# Autodesk Inventor assembly: Robot
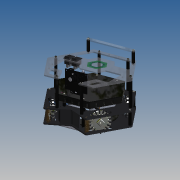
[picture p0: Inventor's stored thumbnail of the model, 180x180]
Saved by Autodesk Inventor 2017 (Build 210142000, 142)
## iProperties
Created: 2016-10-01
Part Number: Robot
Document SubType Name: Assembly
Designer: James Yelland
Author: James Yelland
## Documents named in this file (33)
- C:\Users\yella\git\LJ-STAND\Design\Models\Robot\Robot.iam
- C:\Users\yella\git\LJ-STAND\Design\Models\Robot\Bottom Plate.ipt
- C:\Users\yella\git\LJ-STAND\Design\Models\Robot\Motor Mount.ipt
- C:\Users\yella\git\LJ-STAND\Design\Models\Fasteners\Standoff 30 F-F.ipt
- C:\Users\yella\git\LJ-STAND\Design\Models\Fasteners\M3x10 Screw.ipt
- C:\Users\yella\git\LJ-STAND\Design\Models\Fasteners\M3 Hex Nut.ipt
- C:\Users\yella\git\LJ-STAND\Design\Models\Common\Imported Components\maxon_PN_0_1\maxon_PN_0_1.iam
- C:\Users\yella\git\LJ-STAND\Design\Models\Fasteners\M2x4 Screw.ipt
- C:\Users\yella\git\LJ-STAND\Design\Models\Robot\Light Sensor PCB.ipt
- C:\Users\yella\git\LJ-STAND\Design\Models\Common\Wheel.ipt
- C:\Users\yella\git\LJ-STAND\Design\Models\Robot\Middle Plate.ipt
- C:\Users\yella\git\LJ-STAND\Design\Models\Robot\TSOP Cover Ring.ipt
- C:\Users\yella\git\LJ-STAND\Design\Models\Robot\Main PCB.ipt
- C:\Users\yella\git\LJ-STAND\Design\Models\Fasteners\M3x20 Screw.ipt
- C:\Users\yella\git\LJ-STAND\Design\Models\Common\Pixy angle bracket.ipt
- C:\Users\yella\git\LJ-STAND\Design\Models\Pixy\pixy\Imported Components\Pixy(CMUcam5)\Pixy(CMUcam5).iam
- C:\Users\yella\git\LJ-STAND\Design\Models\Fasteners\Standoff 65 M-F.ipt
- C:\Users\yella\git\LJ-STAND\Design\Models\Robot\Top Plate.ipt
- C:\Users\yella\git\LJ-STAND\Design\Models\Robot\Handle.ipt
- C:\Users\yella\git\LJ-STAND\Design\Models\Common\Rocker switch.ipt
- C:\Users\yella\git\LJ-STAND\Design\Models\Fasteners\Standoff 25 F-F.ipt
- C:\Users\yella\git\LJ-STAND\Design\Models\Robot\Sonar Mount.ipt
- C:\Users\yella\git\LJ-STAND\Design\Models\Fasteners\M3x6 Screw.ipt
- C:\Users\yella\git\LJ-STAND\Design\Models\Common\Sonar.ipt
- C:\Users\yella\git\LJ-STAND\Design\Models\Robot\Light Sensor Cover.ipt
- C:\Users\yella\git\LJ-STAND\Design\Models\Robot\Motor sleeve.ipt
- C:\Users\yella\git\LJ-STAND\Design\Models\Robot\Laser Mount Plate.ipt
- C:\Users\yella\git\LJ-STAND\Design\Models\Robot\LDR Mount Plate.ipt
- C:\Users\yella\git\LJ-STAND\Design\Models\Robot\Light gate compression plate.ipt
- C:\Users\yella\git\LJ-STAND\Design\Models\Fasteners\Standoff 10 M-F.ipt
- C:\Users\yella\git\LJ-STAND\Design\Models\Common\XBee mount.ipt
- C:\Users\yella\git\LJ-STAND\Design\Models\Robot\Light sensor ball guard.ipt
- C:\Users\yella\git\LJ-STAND\Design\Models\Robot\Ball Capture Zone Cover.ipt
## Components (118 placed, 32 different names)
1. Bottom Plate:1 — Insert:1, Insert:2, Insert:3, Insert:4, Insert:5, Insert:6, Insert:7, Insert:8, Insert:35, Insert:36, Insert:37, Insert:38, Insert:39, Insert:40, Mate:27, Mate:28, Mate:29, Mate:30, Mate:31, Mate:32, Mate:33, Mate:34, Mate:35, Mate:36, Mate:37, Mate:38, Mate:40, Mate:41, Mate:42, Mate:43, Mate:44, Mate:45, Insert:197, Insert:198, Insert:199, Insert:206, Insert:207, Insert:208, Insert:209
2. Motor Mount:1 — Insert:15, Mate:13, Insert:25, Insert:26, Insert:27, Mate:33, Mate:34, Mate:35
3. Motor Mount:2 — Insert:16, Mate:14, Insert:22, Insert:23, Insert:24, Mate:27, Mate:28, Mate:29
4. Motor Mount:3 — Insert:18, Mate:15, Insert:19, Insert:20, Insert:21, Mate:36, Mate:37, Mate:38
5. Motor Mount:4 — Insert:17, Mate:16, Insert:28, Insert:29, Insert:30, Mate:30, Mate:31, Mate:32
6. Standoff 30 F-F:1 — Insert:3
7. Standoff 30 F-F:2 — Insert:4
8. Standoff 30 F-F:3 — Insert:2, Insert:50, Insert:127
9. Standoff 30 F-F:4 — Insert:1, Insert:49, Insert:126
10. M3x10 Screw:1 — Insert:5
11. M3x10 Screw:2 — Insert:7
12. M3x10 Screw:3 — Insert:6
13. M3x10 Screw:4 — Insert:8
14. maxon_PN_0_1:1 [sub-assembly] — Insert:16, Mate:14, Mate:18, Flush:2, Insert:184, Angle:3
15. maxon_PN_0_1:2 [sub-assembly] — Insert:17, Mate:16, Mate:20, Flush:4
16. maxon_PN_0_1:3 [sub-assembly] — Insert:15, Mate:13, Mate:19, Flush:3
17. maxon_PN_0_1:4 [sub-assembly] — Insert:18, Mate:15, Mate:17, Flush:1
18. M2x4 Screw:1 — Insert:25
19. M2x4 Screw:3 — Insert:19
20. M2x4 Screw:4 — Insert:28
21. M2x4 Screw:5 — Insert:27
22. M2x4 Screw:6 — Insert:26
23. M2x4 Screw:7 — Insert:24
24. M2x4 Screw:8 — Insert:21
25. M2x4 Screw:9 — Insert:20
26. M2x4 Screw:10 — Insert:29
27. M2x4 Screw:11 — Insert:23
28. M2x4 Screw:12 — Insert:22
29. M2x4 Screw:13 — Insert:30
30. Light Sensor PCB:1 — Insert:35, Insert:36, Insert:41, Insert:42, Insert:43, Insert:44
31. M3 Hex Nut:3 — Insert:41
32. M3x10 Screw:7 — Insert:37
33. M3 Hex Nut:4 — Insert:42, Insert:182
34. M3x10 Screw:8 — Insert:38
35. M3 Hex Nut:5 — Insert:43, Insert:183
36. M3x10 Screw:9 — Insert:39
37. M3 Hex Nut:6 — Insert:44
38. M3x10 Screw:10 — Insert:40
39. Wheel:1 — Mate:18, Flush:2
40. Wheel:2 — Mate:19, Flush:3
41. Wheel:3 — Mate:17, Flush:1
42. Wheel:4 — Mate:20, Flush:4
43. Middle Plate:1 — Insert:49, Insert:50, Insert:102, Insert:103, Insert:104, Insert:105, Insert:106, Insert:107, Insert:120, Insert:121, Insert:122, Insert:123, Insert:124, Insert:125, Insert:126, Insert:127, Insert:128, Insert:129, Insert:130, Insert:131, Insert:191, Insert:192, Insert:193, Insert:194
44. TSOP Cover Ring:1 — Insert:69, Insert:70, Angle:1, Angle:2, Insert:195, Insert:196
45. Main PCB:1 — Insert:69, Insert:70, Insert:71, Insert:72, Insert:73, Insert:74, Insert:94, Insert:95
46. M3x20 Screw:1 — Insert:74
47. M3x20 Screw:2 — Insert:73
48. M3x20 Screw:3 — Insert:72
49. M3x20 Screw:4 — Insert:71
50. Pixy angle bracket:1 — Insert:95, Angle:2, Insert:168
51. Pixy angle bracket:2 — Insert:94, Angle:1, Insert:169
52. Pixy(CMUcam5):1 [sub-assembly] — Insert:168, Insert:169
53. Standoff 65 M-F:3 — Insert:102
54. Standoff 65 M-F:4 — Insert:103, Insert:140
55. Standoff 65 M-F:5 — Insert:106
56. Standoff 65 M-F:6 — Insert:107
57. Standoff 65 M-F:7 — Insert:105, Insert:141
58. Standoff 65 M-F:8 — Insert:104
59. Handle:1 — Insert:136, Insert:137, Insert:138, Insert:139
60. M3x10 Screw:19 — Insert:120
61. M3x10 Screw:20 — Insert:122
62. M3 Hex Nut:17 — Insert:146
63. M3x10 Screw:21 — Insert:125
64. M3 Hex Nut:18 — Insert:144
65. M3x10 Screw:22 — Insert:124
66. M3 Hex Nut:19 — Insert:151
67. M3x10 Screw:23 — Insert:123
68. M3 Hex Nut:20 — Insert:150
69. M3x10 Screw:24 — Insert:121
70. Rocker switch:1 — Mate:21, Mate:22, Mate:23
71. Rocker switch:2 — Mate:24, Mate:25, Mate:26
72. M3x10 Screw:25 — Insert:131
73. M3x10 Screw:26 — Insert:130
74. M3x10 Screw:27 — Insert:129
75. M3x10 Screw:28 — Insert:128
76. Standoff 25 F-F:1 — Insert:137, Insert:143
77. Standoff 25 F-F:2 — Insert:136, Insert:142
78. M3x10 Screw:29 — Insert:149
79. M3x10 Screw:30 — Insert:145
80. M3x10 Screw:31 — Insert:139
81. M3x10 Screw:32 — Insert:138
82. M3 Hex Nut:21 — Insert:147
83. M3 Hex Nut:22 — Insert:148
84. Sonar Mount:1 — Insert:156, Insert:157, Insert:170, Insert:171
85. Sonar Mount:2 — Insert:158, Insert:159, Insert:172, Insert:173
86. Sonar Mount:3 — Insert:152, Insert:153, Insert:176, Insert:177
87. Sonar Mount:4 — Insert:154, Insert:155, Insert:174, Insert:175
88. Top Plate:1 — Insert:140, Insert:141, Insert:142, Insert:143, Insert:144, Insert:145, Insert:146, Insert:147, Insert:148, Insert:149, Insert:150, Insert:151, Insert:152, Insert:153, Insert:154, Insert:155, Mate:21, Mate:22, Mate:23, Mate:24, Mate:25, Mate:26, Insert:156, Insert:157, Insert:158, Insert:159, Insert:160, Insert:161, Insert:162, Insert:163, Insert:164, Insert:165, Insert:166, Insert:167
89. M3x6 Screw:1 — Insert:160
90. M3x6 Screw:2 — Insert:161
91. M3x6 Screw:3 — Insert:162
92. M3x6 Screw:4 — Insert:167
93. M3x6 Screw:5 — Insert:163
94. M3x6 Screw:6 — Insert:165
95. M3x6 Screw:7 — Insert:166
96. M3x6 Screw:8 — Insert:164
97. Sonar:1 — Insert:176, Insert:177
98. Sonar:2 — Insert:174, Insert:175
99. Sonar:3 — Insert:172, Insert:173
100. Sonar:4 — Insert:170, Insert:171
101. Light Sensor Cover:1 — Insert:182, Insert:183
102. Motor sleeve:1 — Insert:184, Angle:3
103. Laser Mount Plate:1 — Mate:40, Mate:41, Mate:42, Insert:185, Insert:186
104. LDR Mount Plate:1 — Mate:43, Mate:44, Mate:45, Insert:187, Insert:188
105. Light gate compression plate:1 — Insert:185, Insert:186
106. Light gate compression plate:2 — Insert:187, Insert:188
107. Standoff 10 M-F:1 — Insert:191, Insert:196
108. Standoff 10 M-F:2 — Insert:194
109. Standoff 10 M-F:3 — Insert:193
110. Standoff 10 M-F:4 — Insert:192, Insert:195
111. XBee mount:1 — Insert:200, Insert:201
112. Standoff 10 M-F:5 — Insert:197, Insert:201
113. Standoff 10 M-F:6 — Insert:199
114. Standoff 10 M-F:7 — Insert:198, Insert:200
115. Standoff 25 F-F:3
116. Standoff 25 F-F:4
117. Light sensor ball guard:1 — Insert:206, Insert:207
118. Ball Capture Zone Cover:1 — Insert:208, Insert:209
## Relationships (165: Insert 126, Mate 32, Flush 4, Angle 3)
- Insert:1: Bottom Plate:1 ↔ Standoff 30 F-F:4
- Insert:2: Bottom Plate:1 ↔ Standoff 30 F-F:3
- Insert:3: Bottom Plate:1 ↔ Standoff 30 F-F:1
- Insert:4: Bottom Plate:1 ↔ Standoff 30 F-F:2
- Insert:5: Bottom Plate:1 ↔ M3x10 Screw:1
- Insert:6: Bottom Plate:1 ↔ M3x10 Screw:3
- Insert:7: Bottom Plate:1 ↔ M3x10 Screw:2
- Insert:8: Bottom Plate:1 ↔ M3x10 Screw:4
- Insert:15: Motor Mount:1 ↔ maxon_PN_0_1:3
- Insert:16: Motor Mount:2 ↔ maxon_PN_0_1:1
- Insert:17: Motor Mount:4 ↔ maxon_PN_0_1:2
- Insert:18: Motor Mount:3 ↔ maxon_PN_0_1:4
- Mate:13: Motor Mount:1 ↔ maxon_PN_0_1:3
- Mate:14: Motor Mount:2 ↔ maxon_PN_0_1:1
- Mate:15: Motor Mount:3 ↔ maxon_PN_0_1:4
- Mate:16: Motor Mount:4 ↔ maxon_PN_0_1:2
- Insert:19: Motor Mount:3 ↔ M2x4 Screw:3
- Insert:20: Motor Mount:3 ↔ M2x4 Screw:9
- Insert:21: Motor Mount:3 ↔ M2x4 Screw:8
- Insert:22: Motor Mount:2 ↔ M2x4 Screw:12
- Insert:23: Motor Mount:2 ↔ M2x4 Screw:11
- Insert:24: Motor Mount:2 ↔ M2x4 Screw:7
- Insert:25: Motor Mount:1 ↔ M2x4 Screw:1
- Insert:26: Motor Mount:1 ↔ M2x4 Screw:6
- Insert:27: Motor Mount:1 ↔ M2x4 Screw:5
- Insert:28: Motor Mount:4 ↔ M2x4 Screw:4
- Insert:29: Motor Mount:4 ↔ M2x4 Screw:10
- Insert:30: Motor Mount:4 ↔ M2x4 Screw:13
- Insert:35: Bottom Plate:1 ↔ Light Sensor PCB:1
- Insert:36: Bottom Plate:1 ↔ Light Sensor PCB:1
- Insert:37: Bottom Plate:1 ↔ M3x10 Screw:7
- Insert:38: Bottom Plate:1 ↔ M3x10 Screw:8
- Insert:39: Bottom Plate:1 ↔ M3x10 Screw:9
- Insert:40: Bottom Plate:1 ↔ M3x10 Screw:10
- Insert:41: Light Sensor PCB:1 ↔ M3 Hex Nut:3
- Insert:42: Light Sensor PCB:1 ↔ M3 Hex Nut:4
- Insert:43: Light Sensor PCB:1 ↔ M3 Hex Nut:5
- Insert:44: Light Sensor PCB:1 ↔ M3 Hex Nut:6
- Mate:17: maxon_PN_0_1:4 ↔ Wheel:3
- Flush:1 (-7 mm): maxon_PN_0_1:4 ↔ Wheel:3
- Mate:18: maxon_PN_0_1:1 ↔ Wheel:1
- Flush:2 (-7 mm): maxon_PN_0_1:1 ↔ Wheel:1
- Mate:19: maxon_PN_0_1:3 ↔ Wheel:2
- Flush:3 (-7 mm): maxon_PN_0_1:3 ↔ Wheel:2
- Mate:20: maxon_PN_0_1:2 ↔ Wheel:4
- Flush:4 (-7 mm): maxon_PN_0_1:2 ↔ Wheel:4
- Insert:49: Standoff 30 F-F:4 ↔ Middle Plate:1
- Insert:50: Standoff 30 F-F:3 ↔ Middle Plate:1
- Insert:69: TSOP Cover Ring:1 ↔ Main PCB:1
- Insert:70: TSOP Cover Ring:1 ↔ Main PCB:1
- Insert:71: Main PCB:1 ↔ M3x20 Screw:4
- Insert:72: Main PCB:1 ↔ M3x20 Screw:3
- Insert:73: Main PCB:1 ↔ M3x20 Screw:2
- Insert:74: Main PCB:1 ↔ M3x20 Screw:1
- Insert:94: Main PCB:1 ↔ Pixy angle bracket:2
- Insert:95: Main PCB:1 ↔ Pixy angle bracket:1
- Insert:102: Middle Plate:1 ↔ Standoff 65 M-F:3
- Insert:103: Middle Plate:1 ↔ Standoff 65 M-F:4
- Insert:104: Middle Plate:1 ↔ Standoff 65 M-F:8
- Insert:105: Middle Plate:1 ↔ Standoff 65 M-F:7
- Insert:106: Middle Plate:1 ↔ Standoff 65 M-F:5
- Insert:107: Middle Plate:1 ↔ Standoff 65 M-F:6
- Insert:120: Middle Plate:1 ↔ M3x10 Screw:19
- Insert:121: Middle Plate:1 ↔ M3x10 Screw:24
- Insert:122: Middle Plate:1 ↔ M3x10 Screw:20
- Insert:123: Middle Plate:1 ↔ M3x10 Screw:23
- Insert:124: Middle Plate:1 ↔ M3x10 Screw:22
- Insert:125: Middle Plate:1 ↔ M3x10 Screw:21
- Insert:126: Standoff 30 F-F:4 ↔ Middle Plate:1
- Insert:127: Standoff 30 F-F:3 ↔ Middle Plate:1
- Insert:128: Middle Plate:1 ↔ M3x10 Screw:28
- Insert:129: Middle Plate:1 ↔ M3x10 Screw:27
- Insert:130: Middle Plate:1 ↔ M3x10 Screw:26
- Insert:131: Middle Plate:1 ↔ M3x10 Screw:25
- Insert:136: Handle:1 ↔ Standoff 25 F-F:2
- Insert:137: Handle:1 ↔ Standoff 25 F-F:1
- Insert:138: Handle:1 ↔ M3x10 Screw:32
- Insert:139: Handle:1 ↔ M3x10 Screw:31
- Insert:140: Standoff 65 M-F:4 ↔ Top Plate:1
- Insert:141: Standoff 65 M-F:7 ↔ Top Plate:1
- Insert:142: Standoff 25 F-F:2 ↔ Top Plate:1
- Insert:143: Standoff 25 F-F:1 ↔ Top Plate:1
- Insert:144: M3 Hex Nut:18 ↔ Top Plate:1
- Insert:145: M3x10 Screw:30 ↔ Top Plate:1
- Insert:146: M3 Hex Nut:17 ↔ Top Plate:1
- Insert:147: M3 Hex Nut:21 ↔ Top Plate:1
- Insert:148: M3 Hex Nut:22 ↔ Top Plate:1
- Insert:149: M3x10 Screw:29 ↔ Top Plate:1
- Insert:150: M3 Hex Nut:20 ↔ Top Plate:1
- Insert:151: M3 Hex Nut:19 ↔ Top Plate:1
- Insert:152: Sonar Mount:3 ↔ Top Plate:1
- Insert:153: Sonar Mount:3 ↔ Top Plate:1
- Insert:154: Sonar Mount:4 ↔ Top Plate:1
- Insert:155: Sonar Mount:4 ↔ Top Plate:1
- Mate:21: Rocker switch:1 ↔ Top Plate:1
- Mate:22: Rocker switch:1 ↔ Top Plate:1
- Mate:23: Rocker switch:1 ↔ Top Plate:1
- Mate:24: Rocker switch:2 ↔ Top Plate:1
- Mate:25: Rocker switch:2 ↔ Top Plate:1
- Mate:26: Rocker switch:2 ↔ Top Plate:1
- Insert:156: Sonar Mount:1 ↔ Top Plate:1
- Insert:157: Sonar Mount:1 ↔ Top Plate:1
- Insert:158: Sonar Mount:2 ↔ Top Plate:1
- Insert:159: Sonar Mount:2 ↔ Top Plate:1
- Insert:160: Top Plate:1 ↔ M3x6 Screw:1
- Insert:161: Top Plate:1 ↔ M3x6 Screw:2
- Insert:162: Top Plate:1 ↔ M3x6 Screw:3
- Insert:163: Top Plate:1 ↔ M3x6 Screw:5
- Insert:164: Top Plate:1 ↔ M3x6 Screw:8
- Insert:165: Top Plate:1 ↔ M3x6 Screw:6
- Insert:166: Top Plate:1 ↔ M3x6 Screw:7
- Insert:167: Top Plate:1 ↔ M3x6 Screw:4
- Angle:1 (0 deg): TSOP Cover Ring:1 ↔ Pixy angle bracket:2
- Angle:2 (0 deg): TSOP Cover Ring:1 ↔ Pixy angle bracket:1
- Insert:168: Pixy angle bracket:1 ↔ Pixy(CMUcam5):1
- Insert:169: Pixy angle bracket:2 ↔ Pixy(CMUcam5):1
- Insert:170: Sonar Mount:1 ↔ Sonar:4
- Insert:171: Sonar Mount:1 ↔ Sonar:4
- Insert:172: Sonar Mount:2 ↔ Sonar:3
- Insert:173: Sonar Mount:2 ↔ Sonar:3
- Insert:174: Sonar Mount:4 ↔ Sonar:2
- Insert:175: Sonar Mount:4 ↔ Sonar:2
- Insert:176: Sonar Mount:3 ↔ Sonar:1
- Insert:177: Sonar Mount:3 ↔ Sonar:1
- Mate:27: Bottom Plate:1 ↔ Motor Mount:2
- Mate:28: Bottom Plate:1 ↔ Motor Mount:2
- Mate:29: Bottom Plate:1 ↔ Motor Mount:2
- Mate:30: Bottom Plate:1 ↔ Motor Mount:4
- Mate:31: Bottom Plate:1 ↔ Motor Mount:4
- Mate:32: Bottom Plate:1 ↔ Motor Mount:4
- Mate:33: Bottom Plate:1 ↔ Motor Mount:1
- Mate:34: Bottom Plate:1 ↔ Motor Mount:1
- Mate:35: Bottom Plate:1 ↔ Motor Mount:1
- Mate:36: Bottom Plate:1 ↔ Motor Mount:3
- Mate:37: Bottom Plate:1 ↔ Motor Mount:3
- Mate:38: Bottom Plate:1 ↔ Motor Mount:3
- Insert:182: M3 Hex Nut:4 ↔ Light Sensor Cover:1
- Insert:183: M3 Hex Nut:5 ↔ Light Sensor Cover:1
- Insert:184: maxon_PN_0_1:1 ↔ Motor sleeve:1
- Angle:3 (0 deg): maxon_PN_0_1:1 ↔ Motor sleeve:1
- Mate:40: Bottom Plate:1 ↔ Laser Mount Plate:1
- Mate:41: Bottom Plate:1 ↔ Laser Mount Plate:1
- Mate:42: Bottom Plate:1 ↔ Laser Mount Plate:1
- Insert:185 (1 mm): Laser Mount Plate:1 ↔ Light gate compression plate:1
- Insert:186 (1 mm): Laser Mount Plate:1 ↔ Light gate compression plate:1
- Mate:43: Bottom Plate:1 ↔ LDR Mount Plate:1
- Mate:44: Bottom Plate:1 ↔ LDR Mount Plate:1
- Mate:45: Bottom Plate:1 ↔ LDR Mount Plate:1
- Insert:187 (1 mm): LDR Mount Plate:1 ↔ Light gate compression plate:2
- Insert:188 (1 mm): LDR Mount Plate:1 ↔ Light gate compression plate:2
- Insert:191: Middle Plate:1 ↔ Standoff 10 M-F:1
- Insert:192: Middle Plate:1 ↔ Standoff 10 M-F:4
- Insert:193: Middle Plate:1 ↔ Standoff 10 M-F:3
- Insert:194: Middle Plate:1 ↔ Standoff 10 M-F:2
- Insert:195: TSOP Cover Ring:1 ↔ Standoff 10 M-F:4
- Insert:196: TSOP Cover Ring:1 ↔ Standoff 10 M-F:1
- Insert:197: Bottom Plate:1 ↔ Standoff 10 M-F:5
- Insert:198: Bottom Plate:1 ↔ Standoff 10 M-F:7
- Insert:199: Bottom Plate:1 ↔ Standoff 10 M-F:6
- Insert:200: XBee mount:1 ↔ Standoff 10 M-F:7
- Insert:201: XBee mount:1 ↔ Standoff 10 M-F:5
- Insert:206: Bottom Plate:1 ↔ Light sensor ball guard:1
- Insert:207: Bottom Plate:1 ↔ Light sensor ball guard:1
- Insert:208: Bottom Plate:1 ↔ Ball Capture Zone Cover:1
- Insert:209: Bottom Plate:1 ↔ Ball Capture Zone Cover:1
